# Autodesk Inventor assembly: Rack
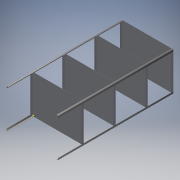
[picture p0: Inventor's stored thumbnail of the model, 180x180]
Saved by Autodesk Inventor 2017 (Build 210142000, 142)
## iProperties
Part Number: Rack
Material: Типовые
Document SubType Name: Assembly
Designer: CAD_Admin
Author: CAD_Admin
## Documents named in this file (3)
- C:\Users\CAD_Admin\AGV 1 computer\AGV_v_0_1_Nastyas_diploma\rack\Rack.iam
- C:\Users\CAD_Admin\AGV 1 computer\AGV_v_0_1_Nastyas_diploma\rack\Угол 32x25x2-1800 ГОСТ 19772-93.ipt
- C:\Users\CAD_Admin\AGV 1 computer\AGV_v_0_1_Nastyas_diploma\rack\Полка.ipt
## Components (8 placed, 2 different names)
1. Угол 32x25x2-1800 ГОСТ 19772-93:1 — Заподлицо:2, Заподлицо:3, Заподлицо:5, Заподлицо:6
2. Угол 32x25x2-1800 ГОСТ 19772-93:2 — Заподлицо:1, Заподлицо:3, Заподлицо:4, Заподлицо:5, Совмещение:5
3. Угол 32x25x2-1800 ГОСТ 19772-93:3 — Заподлицо:2, Заподлицо:6, Заподлицо:7, Совмещение:1, Совмещение:2
4. Угол 32x25x2-1800 ГОСТ 19772-93:4 — Заподлицо:1, Заподлицо:4, Заподлицо:7, Совмещение:3, Совмещение:4, Заподлицо:8
5. Полка:1 — Совмещение:1, Совмещение:2, Совмещение:3, Совмещение:4, Совмещение:5, Заподлицо:8, Заподлицо:9, Заподлицо:10, Заподлицо:11
6. Полка:2 — Заподлицо:9, Заподлицо:10, Заподлицо:11, Заподлицо:12, Заподлицо:13, Заподлицо:14
7. Полка:3 — Заподлицо:12, Заподлицо:13, Заподлицо:14, Заподлицо:15, Заподлицо:16, Заподлицо:17
8. Полка:4 — Заподлицо:15, Заподлицо:16, Заподлицо:17
## Relationships (22: Flush 17, Mate 5)
- Заподлицо:1 [Flush]: Угол 32x25x2-1800 ГОСТ 19772-93:2 ↔ Угол 32x25x2-1800 ГОСТ 19772-93:4
- Заподлицо:2 [Flush]: Угол 32x25x2-1800 ГОСТ 19772-93:1 ↔ Угол 32x25x2-1800 ГОСТ 19772-93:3
- Заподлицо:3 [Flush]: Угол 32x25x2-1800 ГОСТ 19772-93:1 ↔ Угол 32x25x2-1800 ГОСТ 19772-93:2
- Заподлицо:4 [Flush]: Угол 32x25x2-1800 ГОСТ 19772-93:2 ↔ Угол 32x25x2-1800 ГОСТ 19772-93:4
- Заподлицо:5 [Flush]: Угол 32x25x2-1800 ГОСТ 19772-93:1 ↔ Угол 32x25x2-1800 ГОСТ 19772-93:2
- Заподлицо:6 [Flush]: Угол 32x25x2-1800 ГОСТ 19772-93:1 ↔ Угол 32x25x2-1800 ГОСТ 19772-93:3
- Заподлицо:7 [Flush]: Угол 32x25x2-1800 ГОСТ 19772-93:3 ↔ Угол 32x25x2-1800 ГОСТ 19772-93:4
- Совмещение:1 [Mate]: Угол 32x25x2-1800 ГОСТ 19772-93:3 ↔ Полка:1
- Совмещение:2 [Mate]: Угол 32x25x2-1800 ГОСТ 19772-93:3 ↔ Полка:1
- Совмещение:3 [Mate]: Угол 32x25x2-1800 ГОСТ 19772-93:4 ↔ Полка:1
- Совмещение:4 [Mate]: Угол 32x25x2-1800 ГОСТ 19772-93:4 ↔ Полка:1
- Совмещение:5 [Mate]: Угол 32x25x2-1800 ГОСТ 19772-93:2 ↔ Полка:1
- Заподлицо:8 [Flush] (400 mm): Угол 32x25x2-1800 ГОСТ 19772-93:4 ↔ Полка:1
- Заподлицо:9 [Flush]: Полка:1 ↔ Полка:2
- Заподлицо:10 [Flush]: Полка:1 ↔ Полка:2
- Заподлицо:11 [Flush] (-500 mm): Полка:1 ↔ Полка:2
- Заподлицо:12 [Flush]: Полка:2 ↔ Полка:3
- Заподлицо:13 [Flush] (-500 mm): Полка:2 ↔ Полка:3
- Заподлицо:14 [Flush]: Полка:2 ↔ Полка:3
- Заподлицо:15 [Flush] (-400 mm): Полка:3 ↔ Полка:4
- Заподлицо:16 [Flush]: Полка:3 ↔ Полка:4
- Заподлицо:17 [Flush]: Полка:3 ↔ Полка:4
